# Autodesk Inventor assembly: wheel & axil
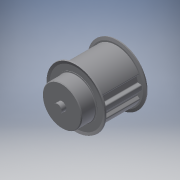
[picture p0: Inventor's stored thumbnail of the model, 180x180]
Saved by Autodesk Inventor 2016 (Build 200138000, 138)
## iProperties
Created: 2015-10-14
Part Number: wheel & axil
Document SubType Name: Assembly
Designer: Delta
Author: Delta
## Documents named in this file (3)
- C:\Robotics\2015-16_CAD\custom cad parts\wheel & axil.iam
- C:\Robotics\2015-16_CAD\COTSParts\Brecoflex\ls40t10_12-2_hub-28x10_d-6h7.ipt
- C:\Robotics\2015-16_CAD\custom cad parts\6mm axil.ipt
## Components (2 placed, 2 different names)
1. ls40t10_12-2_hub-28x10_d-6h7:1 — Mate:1, Flush:1
2. 6mm axil:1 — Mate:1, Flush:1
## Relationships (2: Mate 1, Flush 1)
- Mate:1: ls40t10_12-2_hub-28x10_d-6h7:1 ↔ 6mm axil:1
- Flush:1 (3.175 mm): ls40t10_12-2_hub-28x10_d-6h7:1 ↔ 6mm axil:1
